# Autodesk Inventor assembly: GE-20100_1
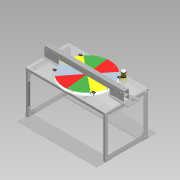
[picture p0: Inventor's stored thumbnail of the model, 180x180]
Saved by Autodesk Inventor 2020.1 (Build 241239000, 239)
## iProperties
Created: 2019-10-14
Part Number: GE-20100_1
Document SubType Name: Assembly
Designer: Phillips Lenovo
Author: Phillips Lenovo
Revision Number: ANY
## Documents named in this file (34)
- D:\FIRST 2020\FRC 2020\FRC Field 2020\Parts\GE-20100_1.iam
- D:\FIRST 2020\FRC 2020\FRC Field 2020\Parts\GE-20102_1.iam
- D:\FIRST 2020\FRC 2020\FRC Field 2020\Parts\GE-20101_2.iam
- D:\FIRST 2020\FRC 2020\FRC Field 2020\Parts\GE-20101_3.iam
- D:\FIRST 2020\FRC 2020\FRC Field 2020\Parts\GE-20114.ipt
- D:\FIRST 2020\FRC 2020\FRC Field 2020\Parts\GE-20104_1.iam
- D:\FIRST 2020\FRC 2020\FRC Field 2020\Parts\GE-20115.ipt
- D:\FIRST 2020\FRC 2020\FRC Field 2020\Parts\am-0516 0.375'''' id bearing, shielded (R6ZZ).step.ipt
- D:\FIRST 2020\FRC 2020\FRC Field 2020\Parts\GE-20121.ipt
- D:\FIRST 2020\FRC 2020\FRC Field 2020\Parts\91255A617_ALLOY STEEL BUTTON-HEAD SOCKET CAP SCREW_91255A617.ipt
- D:\FIRST 2020\FRC 2020\FRC Field 2020\Parts\92511A109_ALUM UNTHRD SPACER_92511A109.ipt
- D:\FIRST 2020\FRC 2020\FRC Field 2020\Parts\855t-bpm10.ipt
- D:\FIRST 2020\FRC 2020\FRC Field 2020\Parts\91253A540_ALLOY STEEL FLAT-HEAD SOCKET CAP SCREW_91253A540.ipt
- D:\FIRST 2020\FRC 2020\FRC Field 2020\Parts\92949A267_18-8 SS BUTTON HEAD HEX DRIVE SCREW_92949A267.ipt
- D:\FIRST 2020\FRC 2020\FRC Field 2020\Parts\91253A550_ALLOY STEEL FLAT-HEAD SOCKET CAP SCREW_91253A550.ipt
- D:\FIRST 2020\FRC 2020\FRC Field 2020\Parts\GE-20140_hinged top_1.iam
- D:\FIRST 2020\FRC 2020\FRC Field 2020\Parts\90985A126_HIGH PROFILE PUSH-BUTTON QUICK-RELEASE PIN_90985A126.ipt
- D:\FIRST 2020\FRC 2020\FRC Field 2020\Parts\GE-20123.ipt
- D:\FIRST 2020\FRC 2020\FRC Field 2020\Parts\GE-20141.ipt
- D:\FIRST 2020\FRC 2020\FRC Field 2020\Parts\46CLR.stp.ipt
- D:\FIRST 2020\FRC 2020\FRC Field 2020\Parts\GE-20142.ipt
- D:\FIRST 2020\FRC 2020\FRC Field 2020\Parts\GE-20143.ipt
- D:\FIRST 2020\FRC 2020\FRC Field 2020\Parts\90272A835_ZINC-PLTD STL PAN HEAD PHILLIPS MACHINE SCREW_90272A835.ipt
- D:\FIRST 2020\FRC 2020\FRC Field 2020\Parts\90631A411_LOW-STRENGTH STEEL NYLON-INSERT LOCKNUT_90631A411.ipt
- D:\FIRST 2020\FRC 2020\FRC Field 2020\Parts\GE-20150_1.iam
- D:\FIRST 2020\FRC 2020\FRC Field 2020\Parts\95615A120_ZINC-PLATED GRADE 5 STL NYLON-INSERT LOCKNUT_95615A120.ipt
- D:\FIRST 2020\FRC 2020\FRC Field 2020\Parts\95615A140_ZINC-PLATED GRADE 5 STL NYLON-INSERT LOCKNUT_95615A140.ipt
- D:\FIRST 2020\FRC 2020\FRC Field 2020\Parts\Hook_1_15.ipt
- D:\FIRST 2020\FRC 2020\FRC Field 2020\Parts\Loop_1_15.ipt
- D:\FIRST 2020\FRC 2020\FRC Field 2020\Parts\Hook_4_55.ipt
- D:\FIRST 2020\FRC 2020\FRC Field 2020\Parts\855t_module_2.iam
- D:\FIRST 2020\FRC 2020\FRC Field 2020\Parts\855t_module_3.iam
- D:\FIRST 2020\FRC 2020\FRC Field 2020\Parts\855T-CAP.ipt
- 46CLR.stp
## Components (144 placed, 144 different names)
1. GE-20102_2172 [sub-assembly]
2. GE-20101_2173 [sub-assembly]
3. GE-20101_2174 [sub-assembly]
4. GE-20114_2175
5. GE-20104_2176 [sub-assembly] — Insert:1, Rotational:1
6. GE-20115_2177
7. GE-20115_2178
8. am-0516 0.375'''' id bearing, shielded (R6ZZ).step_2179
9. am-0516 0.375'''' id bearing, shielded (R6ZZ).step_2180
10. am-0516 0.375'''' id bearing, shielded (R6ZZ).step_2181
11. am-0516 0.375'''' id bearing, shielded (R6ZZ).step_2182
12. am-0516 0.375'''' id bearing, shielded (R6ZZ).step_2183
13. am-0516 0.375'''' id bearing, shielded (R6ZZ).step_2184
14. am-0516 0.375'''' id bearing, shielded (R6ZZ).step_2185
15. am-0516 0.375'''' id bearing, shielded (R6ZZ).step_2186
16. GE-20121_2187
17. GE-20121_2188
18. GE-20121_2189
19. GE-20121_2190
20. 91255A617_ALLOY STEEL BUTTON-HEAD SOCKET CAP SCREW_91255A617_2191
21. 92511A109_ALUM UNTHRD SPACER_92511A109_2192
22. 92511A109_ALUM UNTHRD SPACER_92511A109_2193
23. 92511A109_ALUM UNTHRD SPACER_92511A109_2194
24. 91255A617_ALLOY STEEL BUTTON-HEAD SOCKET CAP SCREW_91255A617_2195
25. 91255A617_ALLOY STEEL BUTTON-HEAD SOCKET CAP SCREW_91255A617_2196
26. 91255A617_ALLOY STEEL BUTTON-HEAD SOCKET CAP SCREW_91255A617_2197
27. 855t-bpm10_2198
28. 91253A540_ALLOY STEEL FLAT-HEAD SOCKET CAP SCREW_91253A540_2199
29. 91253A540_ALLOY STEEL FLAT-HEAD SOCKET CAP SCREW_91253A540_2200
30. 91253A540_ALLOY STEEL FLAT-HEAD SOCKET CAP SCREW_91253A540_2201
31. 91253A540_ALLOY STEEL FLAT-HEAD SOCKET CAP SCREW_91253A540_2202
32. 91253A540_ALLOY STEEL FLAT-HEAD SOCKET CAP SCREW_91253A540_2203
33. 91253A540_ALLOY STEEL FLAT-HEAD SOCKET CAP SCREW_91253A540_2204
34. 91253A540_ALLOY STEEL FLAT-HEAD SOCKET CAP SCREW_91253A540_2205
35. 91253A540_ALLOY STEEL FLAT-HEAD SOCKET CAP SCREW_91253A540_2206
36. 92949A267_18-8 SS BUTTON HEAD HEX DRIVE SCREW_92949A267_2207
37. 92949A267_18-8 SS BUTTON HEAD HEX DRIVE SCREW_92949A267_2208
38. 92949A267_18-8 SS BUTTON HEAD HEX DRIVE SCREW_92949A267_2209
39. 92949A267_18-8 SS BUTTON HEAD HEX DRIVE SCREW_92949A267_2210
40. 91253A550_ALLOY STEEL FLAT-HEAD SOCKET CAP SCREW_91253A550_2211
41. 91253A550_ALLOY STEEL FLAT-HEAD SOCKET CAP SCREW_91253A550_2212
42. 91253A550_ALLOY STEEL FLAT-HEAD SOCKET CAP SCREW_91253A550_2213
43. 91253A550_ALLOY STEEL FLAT-HEAD SOCKET CAP SCREW_91253A550_2214
44. GE-20140_hinged top_2215 [sub-assembly]
45. 90985A126_HIGH PROFILE PUSH-BUTTON QUICK-RELEASE PIN_90985A126_2216
46. GE-20123_2217
47. GE-20123_2218
48. GE-20141_2219
49. GE-20141_2220
50. 46CLR.stp_2221
51. GE-20142_2222
52. 90985A126_HIGH PROFILE PUSH-BUTTON QUICK-RELEASE PIN_90985A126_2223
53. 90985A126_HIGH PROFILE PUSH-BUTTON QUICK-RELEASE PIN_90985A126_2224
54. 90985A126_HIGH PROFILE PUSH-BUTTON QUICK-RELEASE PIN_90985A126_2225
55. 92949A267_18-8 SS BUTTON HEAD HEX DRIVE SCREW_92949A267_2226
56. 92949A267_18-8 SS BUTTON HEAD HEX DRIVE SCREW_92949A267_2227
57. 92949A267_18-8 SS BUTTON HEAD HEX DRIVE SCREW_92949A267_2228
58. 92949A267_18-8 SS BUTTON HEAD HEX DRIVE SCREW_92949A267_2229
59. 92949A267_18-8 SS BUTTON HEAD HEX DRIVE SCREW_92949A267_2230
60. 92949A267_18-8 SS BUTTON HEAD HEX DRIVE SCREW_92949A267_2231
61. 92949A267_18-8 SS BUTTON HEAD HEX DRIVE SCREW_92949A267_2232
62. 92949A267_18-8 SS BUTTON HEAD HEX DRIVE SCREW_92949A267_2233
63. 92949A267_18-8 SS BUTTON HEAD HEX DRIVE SCREW_92949A267_2234
64. 92949A267_18-8 SS BUTTON HEAD HEX DRIVE SCREW_92949A267_2235
65. 92949A267_18-8 SS BUTTON HEAD HEX DRIVE SCREW_92949A267_2236
66. 92949A267_18-8 SS BUTTON HEAD HEX DRIVE SCREW_92949A267_2237
67. 92511A109_ALUM UNTHRD SPACER_92511A109_2238
68. GE-20143_2239
69. 90272A835_ZINC-PLTD STL PAN HEAD PHILLIPS MACHINE SCREW_90272A835_2240
70. 90272A835_ZINC-PLTD STL PAN HEAD PHILLIPS MACHINE SCREW_90272A835_2241
71. 90272A835_ZINC-PLTD STL PAN HEAD PHILLIPS MACHINE SCREW_90272A835_2242
72. 90272A835_ZINC-PLTD STL PAN HEAD PHILLIPS MACHINE SCREW_90272A835_2243
73. 90631A411_LOW-STRENGTH STEEL NYLON-INSERT LOCKNUT_90631A411_2244
74. 90631A411_LOW-STRENGTH STEEL NYLON-INSERT LOCKNUT_90631A411_2245
75. 90631A411_LOW-STRENGTH STEEL NYLON-INSERT LOCKNUT_90631A411_2246
76. 90631A411_LOW-STRENGTH STEEL NYLON-INSERT LOCKNUT_90631A411_2247
77. 90631A411_LOW-STRENGTH STEEL NYLON-INSERT LOCKNUT_90631A411_2248
78. 90631A411_LOW-STRENGTH STEEL NYLON-INSERT LOCKNUT_90631A411_2249
79. 90631A411_LOW-STRENGTH STEEL NYLON-INSERT LOCKNUT_90631A411_2250
80. 90631A411_LOW-STRENGTH STEEL NYLON-INSERT LOCKNUT_90631A411_2251
81. 90631A411_LOW-STRENGTH STEEL NYLON-INSERT LOCKNUT_90631A411_2252
82. 90631A411_LOW-STRENGTH STEEL NYLON-INSERT LOCKNUT_90631A411_2253
83. 90631A411_LOW-STRENGTH STEEL NYLON-INSERT LOCKNUT_90631A411_2254
84. 90631A411_LOW-STRENGTH STEEL NYLON-INSERT LOCKNUT_90631A411_2255
85. 90631A411_LOW-STRENGTH STEEL NYLON-INSERT LOCKNUT_90631A411_2256
86. 90631A411_LOW-STRENGTH STEEL NYLON-INSERT LOCKNUT_90631A411_2257
87. 90631A411_LOW-STRENGTH STEEL NYLON-INSERT LOCKNUT_90631A411_2258
88. 90631A411_LOW-STRENGTH STEEL NYLON-INSERT LOCKNUT_90631A411_2259
89. 90631A411_LOW-STRENGTH STEEL NYLON-INSERT LOCKNUT_90631A411_2260
90. 90631A411_LOW-STRENGTH STEEL NYLON-INSERT LOCKNUT_90631A411_2261
91. 90631A411_LOW-STRENGTH STEEL NYLON-INSERT LOCKNUT_90631A411_2262
92. 90631A411_LOW-STRENGTH STEEL NYLON-INSERT LOCKNUT_90631A411_2263
93. 92949A267_18-8 SS BUTTON HEAD HEX DRIVE SCREW_92949A267_2264
94. 92949A267_18-8 SS BUTTON HEAD HEX DRIVE SCREW_92949A267_2265
95. 92949A267_18-8 SS BUTTON HEAD HEX DRIVE SCREW_92949A267_2266
96. 92949A267_18-8 SS BUTTON HEAD HEX DRIVE SCREW_92949A267_2267
97. 92949A267_18-8 SS BUTTON HEAD HEX DRIVE SCREW_92949A267_2268
98. 92949A267_18-8 SS BUTTON HEAD HEX DRIVE SCREW_92949A267_2269
99. 92949A267_18-8 SS BUTTON HEAD HEX DRIVE SCREW_92949A267_2270
100. 92949A267_18-8 SS BUTTON HEAD HEX DRIVE SCREW_92949A267_2271
101. 92949A267_18-8 SS BUTTON HEAD HEX DRIVE SCREW_92949A267_2272
102. 92949A267_18-8 SS BUTTON HEAD HEX DRIVE SCREW_92949A267_2273
103. 92949A267_18-8 SS BUTTON HEAD HEX DRIVE SCREW_92949A267_2274
104. 92949A267_18-8 SS BUTTON HEAD HEX DRIVE SCREW_92949A267_2275
105. 90631A411_LOW-STRENGTH STEEL NYLON-INSERT LOCKNUT_90631A411_2276
106. 90631A411_LOW-STRENGTH STEEL NYLON-INSERT LOCKNUT_90631A411_2277
107. 90631A411_LOW-STRENGTH STEEL NYLON-INSERT LOCKNUT_90631A411_2278
108. 90631A411_LOW-STRENGTH STEEL NYLON-INSERT LOCKNUT_90631A411_2279
109. 90631A411_LOW-STRENGTH STEEL NYLON-INSERT LOCKNUT_90631A411_2280
110. 90631A411_LOW-STRENGTH STEEL NYLON-INSERT LOCKNUT_90631A411_2281
111. 90631A411_LOW-STRENGTH STEEL NYLON-INSERT LOCKNUT_90631A411_2282
112. 90631A411_LOW-STRENGTH STEEL NYLON-INSERT LOCKNUT_90631A411_2283
113. GE-20150_2284 [sub-assembly] — Insert:1, Rotational:1
114. 95615A120_ZINC-PLATED GRADE 5 STL NYLON-INSERT LOCKNUT_95615A120_2285
115. 95615A120_ZINC-PLATED GRADE 5 STL NYLON-INSERT LOCKNUT_95615A120_2286
116. 95615A120_ZINC-PLATED GRADE 5 STL NYLON-INSERT LOCKNUT_95615A120_2287
117. 95615A120_ZINC-PLATED GRADE 5 STL NYLON-INSERT LOCKNUT_95615A120_2288
118. 95615A120_ZINC-PLATED GRADE 5 STL NYLON-INSERT LOCKNUT_95615A120_2289
119. 95615A120_ZINC-PLATED GRADE 5 STL NYLON-INSERT LOCKNUT_95615A120_2290
120. 95615A120_ZINC-PLATED GRADE 5 STL NYLON-INSERT LOCKNUT_95615A120_2291
121. 95615A120_ZINC-PLATED GRADE 5 STL NYLON-INSERT LOCKNUT_95615A120_2292
122. 95615A120_ZINC-PLATED GRADE 5 STL NYLON-INSERT LOCKNUT_95615A120_2293
123. 95615A120_ZINC-PLATED GRADE 5 STL NYLON-INSERT LOCKNUT_95615A120_2294
124. 95615A120_ZINC-PLATED GRADE 5 STL NYLON-INSERT LOCKNUT_95615A120_2295
125. 95615A120_ZINC-PLATED GRADE 5 STL NYLON-INSERT LOCKNUT_95615A120_2296
126. 95615A140_ZINC-PLATED GRADE 5 STL NYLON-INSERT LOCKNUT_95615A140_2297
127. 95615A140_ZINC-PLATED GRADE 5 STL NYLON-INSERT LOCKNUT_95615A140_2298
128. 95615A140_ZINC-PLATED GRADE 5 STL NYLON-INSERT LOCKNUT_95615A140_2299
129. 95615A140_ZINC-PLATED GRADE 5 STL NYLON-INSERT LOCKNUT_95615A140_2300
130. Hook_1_15_2301
131. Hook_1_15_2302
132. Hook_1_15_2303
133. Hook_1_15_2304
134. Loop_1_15_2305
135. Loop_1_15_2306
136. Loop_1_15_2307
137. Loop_1_15_2308
138. Hook_4_55_2309
139. Hook_4_55_2310
140. Hook_4_55_2311
141. Hook_4_55_2312
142. 855t_module_2313 [sub-assembly]
143. 855t_module_2314 [sub-assembly]
144. 855T-CAP_2315
## Relationships (2: Insert 1, RevoluteJoint 1)
- Insert:1 (4.3942 mm): GE-20104_2176 ↔ GE-20150_2284
- Rotational:1 [RevoluteJoint] (80.9625 mm): GE-20104_2176 ↔ GE-20150_2284
